# Autodesk Inventor assembly: FluidDiagram
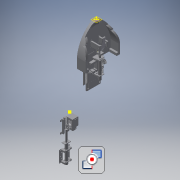
[picture p0: Inventor's stored thumbnail of the model, 180x180]
Saved by Autodesk Inventor 2018 (Build 220112000, 112)
## iProperties
Created: 2018-06-18
Part Number: FluidDiagram
Document SubType Name: Assembly
Designer: reide
Author: reide
## Documents named in this file (18)
- C:\Users\reide\OneDrive\Documents\Inventor\TSA\2018\Animatronics\Tortoise\FluidDiagram.iam
- C:\Users\reide\OneDrive\Documents\Inventor\TSA\2018\Animatronics\Tortoise\Head\HeadBasePt1.iam
- C:\Users\reide\OneDrive\Documents\Inventor\TSA\2018\Animatronics\Tortoise\Head\HeadBottom1.ipt
- C:\Users\reide\OneDrive\Documents\Inventor\TSA\2018\Animatronics\Tortoise\Head\SyringeAttachment.ipt
- C:\Users\reide\OneDrive\Documents\Inventor\TSA\2018\Animatronics\Tortoise\Syringe3mL\SyringEnd.ipt
- C:\Users\reide\OneDrive\Documents\Inventor\TSA\2018\Animatronics\Tortoise\Head\HeadLever.ipt
- C:\Users\reide\OneDrive\Documents\Inventor\TSA\2018\Animatronics\Tortoise\Pinion final.ipt
- C:\Users\reide\OneDrive\Documents\Inventor\TSA\2018\Animatronics\Tortoise\Syringe3mL\SyringeBody.ipt
- C:\Users\reide\OneDrive\Documents\Inventor\TSA\2018\Animatronics\Tortoise\Mock Parts\servo (2)_MIR.ipt
- C:\Users\reide\OneDrive\Documents\Inventor\TSA\2018\Animatronics\Tortoise\Frame\SyringeMotorBase_MIR.ipt
- C:\Users\reide\OneDrive\Documents\Inventor\TSA\2018\Animatronics\Tortoise\Clamps\SyringeServoBaseClamp_MIR.ipt
- C:\Users\reide\OneDrive\Documents\Inventor\TSA\2018\Animatronics\Tortoise\Frame\BaseSyringeRackWall.ipt
- C:\Users\reide\OneDrive\Documents\Inventor\TSA\2018\Animatronics\Tortoise\Clamps\SyringeBaseSlotters.ipt
- C:\Users\reide\OneDrive\Documents\Inventor\TSA\2018\Animatronics\Tortoise\Head\HeadOpenRack.ipt
- C:\Users\reide\OneDrive\Documents\Inventor\TSA\2018\Animatronics\Tortoise\Head\SyringeHeadLeverAttachment.ipt
- C:\Users\reide\OneDrive\Documents\Inventor\TSA\2018\Animatronics\Tortoise\Head\LeverArm.ipt
- C:\Users\reide\OneDrive\Documents\Inventor\TSA\2018\Animatronics\Tortoise\Head\HeadLeverAssemblyAttacher.ipt
- C:\Users\reide\OneDrive\Documents\Inventor\TSA\2018\Animatronics\Tortoise\Head\HeadBottom.ipt
## Components (27 placed, 17 different names)
1. HeadBasePt1:1 [sub-assembly]
2. HeadBottom1:1 — Mate:38
3. SyringeAttachment:1
4. SyringeAttachment:2
5. SyringEnd:1 — Mate:37
6. HeadLever:1
7. Pinion final:1
8. Pinion final:2
9. SyringeBody:1 — Mate:39, Mate:41
10. servo (2)_MIR:1
11. Pinion final:3
12. SyringeMotorBase_MIR:1
13. SyringeServoBaseClamp_MIR:1
14. BaseSyringeRackWall:1
15. SyringeBaseSlotters:1
16. SyringeBaseSlotters:2 — Mate:40, Mate:42
17. HeadOpenRack:1
18. SyringEnd:2
19. SyringeHeadLeverAttachment:1
20. LeverArm:1
21. LeverArm:2
22. HeadLeverAssemblyAttacher:1
23. HeadBottom:1
24. HeadLeverAssemblyAttacher:2
25. SyringeBody:2 — Mate:37, Mate:38
26. SyringeAttachment:3 — Mate:41, Mate:42
27. SyringeAttachment:4 — Mate:39, Mate:40
## Relationships (48: Mate 42, Flush 5, Angle 1)
- [Mate] (0.25 mm): HeadBottom1:1 ↔ SyringeAttachment:2
- [Mate] (0.25 mm): HeadBottom1:1 ↔ SyringeAttachment:1
- [Mate]: HeadBottom1:1 ↔ SyringeAttachment:2
- [Mate] (0.25 mm): HeadBottom1:1 ↔ SyringeAttachment:2
- [Mate] (0.25 mm): HeadBottom1:1 ↔ SyringeAttachment:2
- [Mate]: HeadBottom1:1 ↔ SyringeAttachment:1
- [Mate] (0.25 mm): HeadBottom1:1 ↔ SyringeAttachment:1
- [Mate] (0.25 mm): HeadBottom1:1 ↔ SyringeAttachment:1
- [Mate]: HeadBasePt1:1 ↔ HeadBottom1:1
- [Mate] (1.75 mm): HeadBasePt1:1 ↔ HeadBottom1:1
- [Angle] (0 deg): HeadBasePt1:1 ↔ HeadBottom1:1
- [Mate]: servo (2)_MIR:1 ↔ Pinion final:3
- [Mate]: servo (2)_MIR:1 ↔ Pinion final:3
- [Flush]: SyringeMotorBase_MIR:1 ↔ SyringeServoBaseClamp_MIR:1
- [Flush]: SyringeMotorBase_MIR:1 ↔ SyringeServoBaseClamp_MIR:1
- [Mate]: SyringeMotorBase_MIR:1 ↔ SyringeServoBaseClamp_MIR:1
- [Mate]: servo (2)_MIR:1 ↔ SyringeMotorBase_MIR:1
- [Flush]: servo (2)_MIR:1 ↔ SyringeMotorBase_MIR:1
- [Mate] (0.25 mm): servo (2)_MIR:1 ↔ SyringeMotorBase_MIR:1
- [Mate]: HeadOpenRack:1 ↔ SyringEnd:2
- [Mate]: HeadOpenRack:1 ↔ SyringEnd:2
- [Mate] (0.5 mm): BaseSyringeRackWall:1 ↔ HeadOpenRack:1
- [Mate]: SyringEnd:1 ↔ SyringeHeadLeverAttachment:1
- [Mate]: SyringEnd:1 ↔ SyringeHeadLeverAttachment:1
- [Mate]: SyringeHeadLeverAttachment:1 ↔ LeverArm:1
- [Mate]: SyringeHeadLeverAttachment:1 ↔ LeverArm:1
- [Mate]: HeadLever:1 ↔ LeverArm:1
- [Mate]: SyringeHeadLeverAttachment:1 ↔ LeverArm:2
- [Mate]: SyringeHeadLeverAttachment:1 ↔ LeverArm:2
- [Mate]: HeadLever:1 ↔ LeverArm:2
- [Flush]: HeadBottom1:1 ↔ HeadBottom:1
- [Mate]: HeadBottom1:1 ↔ HeadBottom:1
- [Mate] (0.25 mm): HeadBottom1:1 ↔ HeadBottom:1
- [Mate]: HeadLeverAssemblyAttacher:1 ↔ HeadBottom:1
- [Mate] (0.25 mm): HeadLeverAssemblyAttacher:1 ↔ HeadBottom:1
- [Mate] (0.25 mm): HeadLeverAssemblyAttacher:1 ↔ HeadBottom:1
- [Mate]: HeadBottom:1 ↔ HeadLeverAssemblyAttacher:2
- [Flush]: HeadLeverAssemblyAttacher:1 ↔ HeadLeverAssemblyAttacher:2
- [Mate] (0.25 mm): HeadBottom:1 ↔ HeadLeverAssemblyAttacher:2
- [Mate]: HeadLever:1 ↔ HeadLeverAssemblyAttacher:1
- [Mate] (0.25 mm): HeadLever:1 ↔ HeadLeverAssemblyAttacher:1
- [Mate]: SyringeBody:1 ↔ SyringEnd:2
- Mate:37: SyringEnd:1 ↔ SyringeBody:2
- Mate:38: HeadBottom1:1 ↔ SyringeBody:2
- Mate:39: SyringeBody:1 ↔ SyringeAttachment:4
- Mate:40 (0.25 mm): SyringeBaseSlotters:2 ↔ SyringeAttachment:4
- Mate:41: SyringeBody:1 ↔ SyringeAttachment:3
- Mate:42 (0.25 mm): SyringeBaseSlotters:2 ↔ SyringeAttachment:3
## Named parameters: d418_d399 = 0 mm, d419_d378_d391_d333 = 0 mm, d387_d370 = 0 mm, d388_d374 = 0 mm, d181_d156 = 0.25 mm
